# Autodesk Inventor assembly: Version1
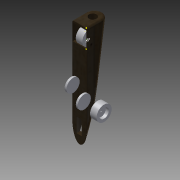
[picture p0: Inventor's stored thumbnail of the model, 180x180]
Saved by Autodesk Inventor 2015 SP2 (Build 190223200, 223)
## iProperties
Created: 2016-04-05
Part Number: Version1
Document SubType Name: Assembly
Designer: cvhssub1
Author: cvhssub1
## Documents named in this file (4)
- U:\Engineering\CO2-Car\Version1.iam
- U:\Engineering\CO2-Car\Car Body 1.ipt
- U:\Engineering\CO2-Car\Front Wheel.ipt
- U:\Engineering\CO2-Car\Back Wheel.ipt
## Components (5 placed, 3 different names)
1. Car Body 1:1 — Mate:1
2. Front Wheel:1
3. Front Wheel:2
4. Back Wheel:1 — Mate:1
5. Back Wheel:2
## Relationships (1: Mate 1)
- Mate:1: Car Body 1:1 ↔ Back Wheel:1
